# Autodesk Inventor assembly: Ensamble
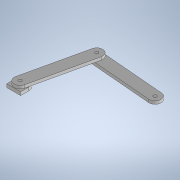
[picture p0: Inventor's stored thumbnail of the model, 180x180]
Saved by Autodesk Inventor 2022 (Build 260153000, 153)
## iProperties
Created: 2022-01-11
Part Number: Ensamble
Document SubType Name: Assembly
Designer: Yeison
Author: Yeison
## Documents named in this file (4)
- C:\Users\Yeison\Documents\GitHub\Servomecanismos\Modelo\Ensamble.iam
- C:\Users\Yeison\Documents\GitHub\Servomecanismos\Modelo\Soporte.ipt
- C:\Users\Yeison\Documents\GitHub\Servomecanismos\Modelo\perno2.ipt
- C:\Users\Yeison\Documents\GitHub\Servomecanismos\Modelo\Eslabon.ipt
## Components (6 placed, 3 different names)
1. Soporte:1 — Rigid:1, Rotational:1
2. perno2:1 — Rigid:1
3. Eslabon:1 — Rotational:1, Rigid:2, Rotational:2
4. perno2:2 — Rigid:2
5. Eslabon:2 — Rotational:2, Rigid:3
6. perno2:3 — Rigid:3
## Relationships (5: WeldJoint 3, RevoluteJoint 2)
- Rigid:1 [WeldJoint]: Soporte:1 ↔ perno2:1
- Rotational:1 [RevoluteJoint]: Soporte:1 ↔ Eslabon:1
- Rigid:2 [WeldJoint]: Eslabon:1 ↔ perno2:2
- Rotational:2 [RevoluteJoint]: Eslabon:1 ↔ Eslabon:2
- Rigid:3 [WeldJoint]: Eslabon:2 ↔ perno2:3
